# Autodesk Inventor assembly: PCBSupport
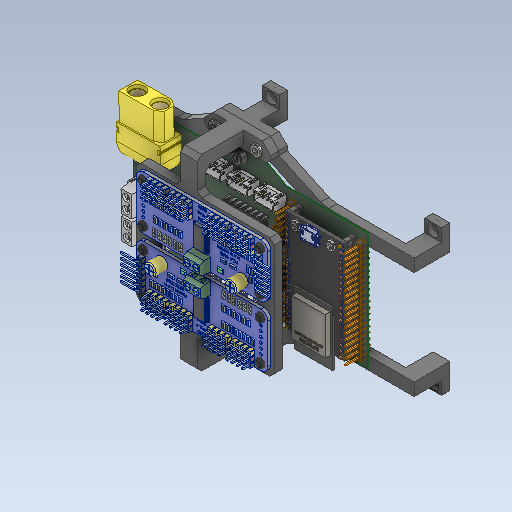
[picture p0: Inventor's stored thumbnail of the model, 512x512]
Saved by Autodesk Inventor 2020 (Build 240168000, 168)
## iProperties
Created: 2021-03-17
Part Number: PCBSupport
Document SubType Name: Assembly
Designer: Turing
Author: Turing
## Documents named in this file (8)
- D:\Hexapod Final Fucking Version\PCBSupport.iam
- D:\Hexapod Final Fucking Version\PCBSupportBot.ipt
- D:\Hexapod Final Fucking Version\PCBSupportTop.ipt
- D:\Hexapod Final Fucking Version\12Channel PWM.ipt
- D:\Hexapod Final Fucking Version\HexaBoard.ipt
- D:\Hexapod Final Fucking Version\PCBSupport\Design Accelerator\Bolted Connection1.iam
- D:\Hexapod Final Fucking Version\PCBSupport\Design Accelerator\Bolted Connection2.iam
- D:\Hexapod Final Fucking Version\PCBSupport\Design Accelerator\Bolted Connection3.iam
## Components (8 placed, 5 different names)
1. PCBSupportBot:1 — Rigid:4, Rigid:5, Mate:6
2. PCBSupportTop:1 — Rigid:4, Rotational:1, Rotational:2, Mate:1, Mate:2
3. 12Channel PWM:1 — Rotational:1, Mate:3, Mate:4
4. 12Channel PWM:2 — Rotational:2
5. HexaBoard:1 — Rigid:5, Mate:5
6. PCB Bolted Connection:1 [sub-assembly] — Mate:1, Mate:2
7. PCB Bolted Connection:2 [sub-assembly] — Mate:3, Mate:4
8. PCB Bolted Connection:3 [sub-assembly] — Mate:5, Mate:6
## Relationships (10: Mate 6, WeldJoint 2, RevoluteJoint 2)
- Rigid:4 [WeldJoint]: PCBSupportBot:1 ↔ PCBSupportTop:1
- Rotational:1 [RevoluteJoint]: PCBSupportTop:1 ↔ 12Channel PWM:1
- Rotational:2 [RevoluteJoint]: PCBSupportTop:1 ↔ 12Channel PWM:2
- Rigid:5 [WeldJoint]: PCBSupportBot:1 ↔ HexaBoard:1
- Mate:1: PCBSupportTop:1 ↔ PCB Bolted Connection:1
- Mate:2: PCBSupportTop:1 ↔ PCB Bolted Connection:1
- Mate:3: 12Channel PWM:1 ↔ PCB Bolted Connection:2
- Mate:4: 12Channel PWM:1 ↔ PCB Bolted Connection:2
- Mate:5: HexaBoard:1 ↔ PCB Bolted Connection:3
- Mate:6: PCBSupportBot:1 ↔ PCB Bolted Connection:3
